# Autodesk Inventor assembly: UpperBody
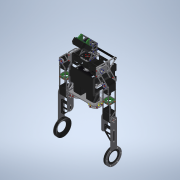
[picture p0: Inventor's stored thumbnail of the model, 180x180]
Saved by Autodesk Inventor 2020.4 (Build 244396000, 396)
## iProperties
Created: 2016-05-03
Part Number: UpperBody
Document SubType Name: Assembly
Designer: hiroaki
Mass: 1684.21 g
Surface Area: 5710.79 cm^2
Volume: 1053.68 cm^3
Density: 1.59841 g/cm^3
Author: hiroaki
## Documents named in this file (9)
- C:\Users\Masato\Documents\Inventor\CIT Brains_Inventor\OpenPlatform_ver3_0 - ve4_1 branch\UpperBody\UpperBody.iam
- C:\Users\Masato\Documents\Inventor\CIT Brains_Inventor\OpenPlatform_ver3_0 - ve4_1 branch\UpperBody\Arm\UpperArm.iam
- C:\Users\Masato\Documents\Inventor\CIT Brains_Inventor\OpenPlatform_ver3_0 - ve4_1 branch\UpperBody\Arm\UpperArm_MIR.iam
- C:\Users\Masato\Documents\Inventor\CIT Brains_Inventor\OpenPlatform_ver3_0 - ve4_1 branch\UpperBody\Head\Head_.iam
- C:\Users\Masato\Documents\Inventor\CIT Brains_Inventor\OpenPlatform_ver3_0 - ve4_1 branch\UpperBody\UpperBody_.iam
- C:\Users\Masato\Documents\Inventor\CIT Brains_Inventor\OpenPlatform_ver3_0 - ve4_1 branch\UpperBody\Cockpit\Cockpit_.iam
- C:\Users\Masato\Documents\Inventor\CIT Brains_Inventor\OpenPlatform_ver3_0 - ve4_1 branch\Ready_Made\Screw\SPNFL-BRN-M3-6.ipt
- C:\Users\Masato\Documents\Inventor\CIT Brains_Inventor\OpenPlatform_ver3_0 - ve4_1 branch\UpperBody\Arm\Shoulder_.iam
- C:\Users\Masato\Documents\Inventor\CIT Brains_Inventor\OpenPlatform_ver3_0 - ve4_1 branch\UpperBody\Arm\ForeArm_.iam
## Components (11 placed, 8 different names)
1. UpperArm_MIR:1 [sub-assembly] — 挿入:113, 角度:35, 挿入:115
2. UpperArm:1 [sub-assembly] — 挿入:111, 角度:34, 挿入:114, 角度:37
3. Head_:1 [sub-assembly] — 挿入:106, 角度:39
4. UpperBody_:1 [sub-assembly] — 挿入:106, フラッシュ:1, フラッシュ:2, フラッシュ:3, 挿入:107, 角度:28, 挿入:108, 挿入:109, 挿入:110, 挿入:112, 角度:36, 角度:39
5. Cockpit_:1 [sub-assembly] — 挿入:107, 角度:28
6. SPNFL-BRN-M3-6:1 — 挿入:108
7. SPNFL-BRN-M3-6:2 — 挿入:109
8. Shoulder_:1 [sub-assembly] — 挿入:110, 挿入:111, 角度:33, 角度:34, 角度:36
9. Shoulder_:2 [sub-assembly] — 挿入:112, 挿入:113, 角度:33, 角度:35
10. ForeArm_:1 [sub-assembly] — 挿入:114, 角度:37, 角度:38
11. ForeArm_:2 [sub-assembly] — 挿入:115, 角度:38
## Relationships (21: Insert 10, Angle 8, Flush 3)
- 挿入:106 [Insert]: Head_:1 ↔ UpperBody_:1
- フラッシュ:1 [Flush]: UpperBody_:1
- フラッシュ:2 [Flush]: UpperBody_:1
- フラッシュ:3 [Flush]: UpperBody_:1
- 挿入:107 [Insert] (0.25 mm): UpperBody_:1 ↔ Cockpit_:1
- 角度:28 [Angle] (0 deg): UpperBody_:1 ↔ Cockpit_:1
- 挿入:108 [Insert]: UpperBody_:1 ↔ SPNFL-BRN-M3-6:1
- 挿入:109 [Insert]: UpperBody_:1 ↔ SPNFL-BRN-M3-6:2
- 挿入:110 [Insert]: UpperBody_:1 ↔ Shoulder_:1
- 挿入:111 [Insert]: UpperArm:1 ↔ Shoulder_:1
- 挿入:112 [Insert]: UpperBody_:1 ↔ Shoulder_:2
- 挿入:113 [Insert]: UpperArm_MIR:1 ↔ Shoulder_:2
- 角度:33 [Angle] (0 deg): Shoulder_:1 ↔ Shoulder_:2
- 角度:34 [Angle] (0 deg): UpperArm:1 ↔ Shoulder_:1
- 角度:35 [Angle] (0 deg): UpperArm_MIR:1 ↔ Shoulder_:2
- 角度:36 [Angle] (0 deg): UpperBody_:1 ↔ Shoulder_:1
- 挿入:114 [Insert]: UpperArm:1 ↔ ForeArm_:1
- 挿入:115 [Insert]: UpperArm_MIR:1 ↔ ForeArm_:2
- 角度:37 [Angle] (0 deg): UpperArm:1 ↔ ForeArm_:1
- 角度:38 [Angle] (0 deg): ForeArm_:1 ↔ ForeArm_:2
- 角度:39 [Angle] (0 deg): Head_:1 ↔ UpperBody_:1
## Named parameters: shoulder_pitch_angle = 0 deg
